# Autodesk Inventor assembly: CAR_012_CarouselDriveAssembly_MIR
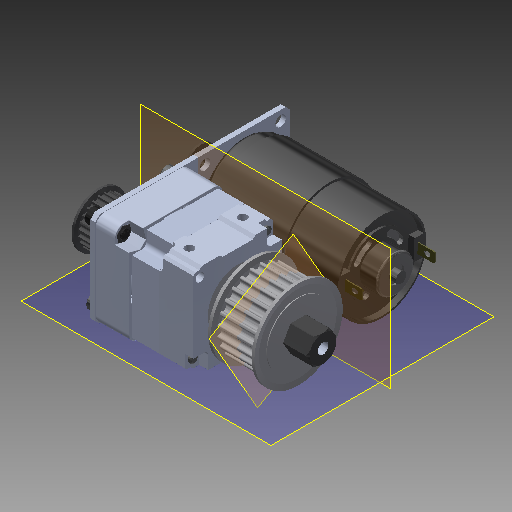
[picture p0: Inventor's stored thumbnail of the model, 512x512]
Saved by Autodesk Inventor 2018 (Build 220112000, 112)
## iProperties
Created: 2020-02-01
Part Number: CAR_012_CarouselDriveAssembly_MIR
Document SubType Name: Assembly
Designer: user
Mass: 787.669 g
Surface Area: 1098.44 cm^2
Volume: 234.441 cm^3
Density: 3.35977 g/cm^3
Author: user
## Documents named in this file (4)
- C:\Users\user\Documents\GrabCAD\New folder\Build season\CAR_012_CarouselDriveAssembly_MIR.iam
- C:\Users\user\Documents\GrabCAD\New folder\Build season\CAR_011_VersaPlanetary_v2_Single_Stage_10_1_with_775_Series_Reverse_MIR.iam
- C:\Users\user\Documents\GrabCAD\New folder\Build season\CHA_007_DrivenPulleyAssembly_MIR1.iam
- C:\Users\user\Documents\GrabCAD\New folder\Build season\CAR_013_24t_x_15mm_Wide_Aluminum_Pulley_HTD_5mm_1_2_Hex_217-4101_MIR.ipt
## Components (3 placed, 3 different names)
1. CAR_011_VersaPlanetary_v2_Single_Stage_10_1_with_775_Series_Reverse_MIR:1 [sub-assembly] — Flush:1, Mate:2, Mate:1, Tangent:1, Angle:1, Mate:5, Mate:4, Mate:3, Tangent:2, Angle:2
2. CHA_007_DrivenPulleyAssembly_MIR1:1 [sub-assembly] — Flush:1, Mate:2, Mate:1
3. CAR_013_24t_x_15mm_Wide_Aluminum_Pulley_HTD_5mm_1_2_Hex_217-4101_MIR:1 — Mate:5, Mate:4, Mate:3
## Relationships (10: Mate 5, Tangent 2, Angle 2, Flush 1)
- Flush:1: CAR_011_VersaPlanetary_v2_Single_Stage_10_1_with_775_Series_Reverse_MIR:1 ↔ CHA_007_DrivenPulleyAssembly_MIR1:1
- Mate:2: CAR_011_VersaPlanetary_v2_Single_Stage_10_1_with_775_Series_Reverse_MIR:1 ↔ CHA_007_DrivenPulleyAssembly_MIR1:1
- Mate:1: CAR_011_VersaPlanetary_v2_Single_Stage_10_1_with_775_Series_Reverse_MIR:1 ↔ CHA_007_DrivenPulleyAssembly_MIR1:1
- Tangent:1: CAR_011_VersaPlanetary_v2_Single_Stage_10_1_with_775_Series_Reverse_MIR:1
- Angle:1 (0 deg): CAR_011_VersaPlanetary_v2_Single_Stage_10_1_with_775_Series_Reverse_MIR:1
- Mate:5 (6.35 mm): CAR_011_VersaPlanetary_v2_Single_Stage_10_1_with_775_Series_Reverse_MIR:1 ↔ CAR_013_24t_x_15mm_Wide_Aluminum_Pulley_HTD_5mm_1_2_Hex_217-4101_MIR:1
- Mate:4: CAR_011_VersaPlanetary_v2_Single_Stage_10_1_with_775_Series_Reverse_MIR:1 ↔ CAR_013_24t_x_15mm_Wide_Aluminum_Pulley_HTD_5mm_1_2_Hex_217-4101_MIR:1
- Mate:3: CAR_011_VersaPlanetary_v2_Single_Stage_10_1_with_775_Series_Reverse_MIR:1 ↔ CAR_013_24t_x_15mm_Wide_Aluminum_Pulley_HTD_5mm_1_2_Hex_217-4101_MIR:1
- Tangent:2: CAR_011_VersaPlanetary_v2_Single_Stage_10_1_with_775_Series_Reverse_MIR:1
- Angle:2 (0 deg): CAR_011_VersaPlanetary_v2_Single_Stage_10_1_with_775_Series_Reverse_MIR:1
